# Autodesk Inventor assembly: Assembly1
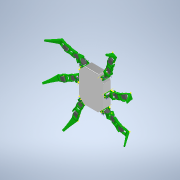
[picture p0: Inventor's stored thumbnail of the model, 180x180]
Saved by Autodesk Inventor 2022 (Build 260153000, 153)
## iProperties
Created: 2022-04-24
Part Number: Assembly1
Document SubType Name: Assembly
Designer: HP
Author: HP
## Documents named in this file (3)
- C:\Users\HP\Documents\Inventor\spider\Assembly1.iam
- C:\Users\HP\Documents\Inventor\spider\body.ipt
- C:\Users\HP\Documents\Inventor\spider\Assembly4.iam
## Components (7 placed, 2 different names)
1. body:1 — Mate:1, Mate:2, Mate:3, Mate:4, Mate:5, Mate:6, Mate:7, Mate:8, Mate:9, Mate:10, Mate:11, Mate:12, Mate:13, Mate:14, Mate:15, Mate:16, Mate:17, Mate:18
2. Assembly4:1 [sub-assembly] — Mate:1, Mate:2, Mate:3
3. Assembly4:2 [sub-assembly] — Mate:4, Mate:5, Mate:6
4. Assembly4:3 [sub-assembly] — Mate:7, Mate:8, Mate:9
5. Assembly4:4 [sub-assembly] — Mate:10, Mate:11, Mate:12
6. Assembly4:5 [sub-assembly] — Mate:13, Mate:14, Mate:15
7. Assembly4:6 [sub-assembly] — Mate:16, Mate:17, Mate:18
## Relationships (18: Mate 18)
- Mate:1: body:1 ↔ Assembly4:1
- Mate:2: body:1 ↔ Assembly4:1
- Mate:3 (90.4748 mm): body:1 ↔ Assembly4:1
- Mate:4: body:1 ↔ Assembly4:2
- Mate:5: body:1 ↔ Assembly4:2
- Mate:6 (87.6808 mm): body:1 ↔ Assembly4:2
- Mate:7: body:1 ↔ Assembly4:3
- Mate:8: body:1 ↔ Assembly4:3
- Mate:9 (17.653 mm): body:1 ↔ Assembly4:3
- Mate:10: body:1 ↔ Assembly4:4
- Mate:11: body:1 ↔ Assembly4:4
- Mate:12 (13.8684 mm): body:1 ↔ Assembly4:4
- Mate:13: body:1 ↔ Assembly4:5
- Mate:14: body:1 ↔ Assembly4:5
- Mate:15 (19.05 mm): body:1 ↔ Assembly4:5
- Mate:16: body:1 ↔ Assembly4:6
- Mate:17: body:1 ↔ Assembly4:6
- Mate:18 (21.5646 mm): body:1 ↔ Assembly4:6
